# Autodesk Inventor assembly: Elevator Gearbox Assembly
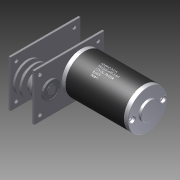
[picture p0: Inventor's stored thumbnail of the model, 180x180]
Saved by Autodesk Inventor 2015 (Build 190159000, 159)
## iProperties
Created: 2015-02-21
Part Number: Elevator Gearbox Assembly
Document SubType Name: Assembly
Designer: szymsea16
Author: szymsea16
## Documents named in this file (9)
- \\lhssvr02\Homedirs\Robotics Club\CAD Model 2015\Elevator parts\Gearbox\Elevator Gearbox Assembly.iam
- \\lhssvr02\Homedirs\Robotics Club\CAD Model 2015\Box Beam Drive Base\Newest\Hex Shaft for E gear box.ipt
- \\lhssvr02\Homedirs\Robotics Club\CAD Model 2015\Elevator parts\Gearbox\Back Gearbox Plate.ipt
- \\lhssvr02\Homedirs\Robotics Club\CAD Model 2015\Elevator parts\Gearbox\Gearbox plate.ipt
- \\lhssvr02\Homedirs\Robotics Club\CAD Model 2015\Parts Folder\Motors\Imported Components\MOT_CIM-Motor_217-2000.iam\FR801-001_CIM Motor Body_MIR2_MIR1.ipt
- \\lhssvr02\Homedirs\Robotics Club\CAD Model 2015\Elevator parts\Gearbox\22 tooth sprocket.ipt
- \\lhssvr02\Homedirs\Robotics Club\CAD Model 2015\Elevator parts\Gearbox\16 tooth sprocket.ipt
- \\lhssvr02\Homedirs\Robotics Club\CAD Model 2015\Elevator parts\Gearbox\Elevator i-sprocket.ipt
- \\lhssvr02\Homedirs\Robotics Club\CAD Model 2015\Box Beam Drive Base\brf-08.ipt
## Components (10 placed, 8 different names)
1. Hex Shaft for E gear box:1 — Mate:4, Mate:5, Mate:6, Mate:10, Flush:4, Flush:5
2. Back Gearbox Plate:2 — Flush:2, Flush:3, Mate:3, Mate:15
3. Gearbox plate:1 — Flush:2, Flush:3, Mate:10, Mate:12, Mate:13
4. FR801-001_CIM Motor Body_MIR2_MIR1:1 — Mate:3, Mate:12, Mate:17
5. 22 tooth sprocket:1 — Mate:6, Mate:8
6. 22 tooth sprocket:2 — Mate:4, Mate:8, Mate:9, Mate:16
7. 16 tooth sprocket:1 — Mate:5, Mate:9, Mate:14
8. Elevator i-sprocket:1 — Mate:17
9. brf-08:1 — Mate:13, Mate:14, Flush:5
10. brf-08:2 — Mate:15, Mate:16, Flush:4
## Relationships (17: Mate 13, Flush 4)
- Flush:2: Back Gearbox Plate:2 ↔ Gearbox plate:1
- Flush:3: Back Gearbox Plate:2 ↔ Gearbox plate:1
- Mate:3: Back Gearbox Plate:2 ↔ FR801-001_CIM Motor Body_MIR2_MIR1:1
- Mate:4: Hex Shaft for E gear box:1 ↔ 22 tooth sprocket:2
- Mate:5: Hex Shaft for E gear box:1 ↔ 16 tooth sprocket:1
- Mate:6: Hex Shaft for E gear box:1 ↔ 22 tooth sprocket:1
- Mate:8: 22 tooth sprocket:1 ↔ 22 tooth sprocket:2
- Mate:9: 22 tooth sprocket:2 ↔ 16 tooth sprocket:1
- Mate:10: Hex Shaft for E gear box:1 ↔ Gearbox plate:1
- Mate:12: Gearbox plate:1 ↔ FR801-001_CIM Motor Body_MIR2_MIR1:1
- Mate:13: Gearbox plate:1 ↔ brf-08:1
- Mate:14: 16 tooth sprocket:1 ↔ brf-08:1
- Mate:15: Back Gearbox Plate:2 ↔ brf-08:2
- Mate:16: 22 tooth sprocket:2 ↔ brf-08:2
- Flush:4: Hex Shaft for E gear box:1 ↔ brf-08:2
- Flush:5: Hex Shaft for E gear box:1 ↔ brf-08:1
- Mate:17: FR801-001_CIM Motor Body_MIR2_MIR1:1 ↔ Elevator i-sprocket:1
